# Autodesk Inventor assembly: 6001JRXZZ
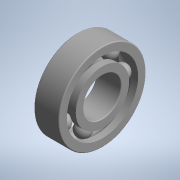
[picture p0: Inventor's stored thumbnail of the model, 180x180]
Saved by Autodesk Inventor 2022.3 (Build 263350000, 350)
## iProperties
Part Number: 6001JRXZZ
Catalog Web Link: www.cadenas.de
Description: Shielded type ZZ-
Vendor: NTN
Document SubType Name: Assembly
Designer: partserver
Manufacturer: NTN
Mass: 2.63039 g
Surface Area: 31.8837 cm^2
Volume: 2.63039 cm^3
Density: 1 g/cm^3
Category: PARTsolutions
Company: NTN
PSOL_IDENT_0: {$CADENAS_DATA\23d-libs\ntn\ball_roller_bearings\deep_groove_bb\deep_groove_bb\dgbb_zz_asmtab.prj},1
PSOL_IDENT_1: 84 {VTYP=3D},{STYP=ASSTAB},{NB=6001JRXZZ},{LINA=6001JRXZZ},{NN=Shielded type ZZ},{DATE=12.08.2020 02
PSOL_IDENT_2: :23:38},{GEOMDATE=29.05.2020 01:04:27},{VERSION=},{LINEID=8380},{WBVAR=},{WBNUMERIC=}  {NB=6001JRXZZ
PSOL_IDENT_3: },{LINA=6001JRXZZ},{KT=DUMMY},{IDNR=},{SD=12},{D=28},{B=8},{R=0.3},{ORDER1=6001JRX},{ORDER=6001JRXZZ
PSOL_IDENT_4: },{CR=5.65},{COR=2.39},{CU=0.3},{CRF=MIN},{CORF=MIN},{LSG=26000},{LSO=30000},{MASS=0.021},{RNS=MIN},
PSOL_IDENT_5: {LLH=MIN},{LLU=MIN},{ST=},{NCST=},{LTST=},{CST=},{SRG=},{SR=},{D1=26.44},{A=2.20},{BA=0.90},{R0=0.30
PSOL_IDENT_6: },{D2=32.7},{F=MIN},{DA1=},{DA2=},{DA=},{DX=MIN},{CY=},{CZ=},{RAS=},{RNAS=0.182},{VERS=2},{X=8},{PPA
PSOL_IDENT_7: TH=dgbb_asmtpl.prj},{RDX=2},{RD=1}
NB: 6001JRXZZ
NN: Shielded type ZZ
NBSYN: $ORDER.
LINA: 6001JRXZZ
CATALOG: NTN Corporation
SD: 12
D: 28
B: 8
R: 0.3
ORDER: 6001JRXZZ
CR: 5.65
COR: 2.39
CU: 0.3
LSG: 26000
LSO: 30000
MASS: 0.021
SUPPLIER: NTN
ARTICLENO: 6001JRXZZ
BOMINFO: 6001JRXZZ
CREATOR: CADENAS GmbH
Title: 6001JRXZZ
Author: Cadenas PARTsolutions
## Documents named in this file (4)
- C:\Users\YusukeKunita\Documents\GrabCAD\Development\BasicParts\Bearing\NTN_6001JRXZZ\6001JRXZZ.iam
- C:\Users\YusukeKunita\Documents\GrabCAD\Development\BasicParts\Bearing\NTN_6001JRXZZ\6001JRX Inner Ring.ipt
- C:\Users\YusukeKunita\Documents\GrabCAD\Development\BasicParts\Bearing\NTN_6001JRXZZ\6001JRX Outer Ring.ipt
- C:\Users\YusukeKunita\Documents\GrabCAD\Development\BasicParts\Bearing\NTN_6001JRXZZ\6001JRX Ball.ipt
## Components (9 placed, 3 different names)
1. 6001JRX Inner Ring:1 — dgbb_ir_XY@1 <-> dgbb_or_XY@2, dgbb_ir_Z@1 <-> dgbb_or_Z@2, dgbb_ir_YZ@1 <-> dgbb_or_YZ@2
2. 6001JRX Outer Ring:1 — dgbb_ir_XY@1 <-> dgbb_or_XY@2, dgbb_ir_Z@1 <-> dgbb_or_Z@2, dgbb_ir_YZ@1 <-> dgbb_or_YZ@2, dgbb_or11_1_XY@2 <-> dgbb_ball_XY@3, dgbb_or11_1_Z@2 <-> dgbb_ball_Z@3, dgbb_or11_1_YZ@2 <-> dgbb_ball_YZ@3, dgbb_or11_2_XY@2 <-> dgbb_ball_XY@4, dgbb_or11_2_Z@2 <-> dgbb_ball_Z@4, dgbb_or11_2_YZ@2 <-> dgbb_ball_YZ@4, dgbb_or11_3_XY@2 <-> dgbb_ball_XY@5, dgbb_or11_3_Z@2 <-> dgbb_ball_Z@5, dgbb_or11_3_YZ@2 <-> dgbb_ball_YZ@5, dgbb_or11_4_XY@2 <-> dgbb_ball_XY@6, dgbb_or11_4_Z@2 <-> dgbb_ball_Z@6, dgbb_or11_4_YZ@2 <-> dgbb_ball_YZ@6, dgbb_or11_5_XY@2 <-> dgbb_ball_XY@7, dgbb_or11_5_Z@2 <-> dgbb_ball_Z@7, dgbb_or11_5_YZ@2 <-> dgbb_ball_YZ@7, dgbb_or11_6_XY@2 <-> dgbb_ball_XY@8, dgbb_or11_6_Z@2 <-> dgbb_ball_Z@8, dgbb_or11_6_YZ@2 <-> dgbb_ball_YZ@8, dgbb_or11_7_XY@2 <-> dgbb_ball_XY@9, dgbb_or11_7_Z@2 <-> dgbb_ball_Z@9, dgbb_or11_7_YZ@2 <-> dgbb_ball_YZ@9
3. 6001JRX Ball:1 — dgbb_or11_1_XY@2 <-> dgbb_ball_XY@3, dgbb_or11_1_Z@2 <-> dgbb_ball_Z@3, dgbb_or11_1_YZ@2 <-> dgbb_ball_YZ@3
4. 6001JRX Ball:2 — dgbb_or11_2_XY@2 <-> dgbb_ball_XY@4, dgbb_or11_2_Z@2 <-> dgbb_ball_Z@4, dgbb_or11_2_YZ@2 <-> dgbb_ball_YZ@4
5. 6001JRX Ball:3 — dgbb_or11_3_XY@2 <-> dgbb_ball_XY@5, dgbb_or11_3_Z@2 <-> dgbb_ball_Z@5, dgbb_or11_3_YZ@2 <-> dgbb_ball_YZ@5
6. 6001JRX Ball:4 — dgbb_or11_4_XY@2 <-> dgbb_ball_XY@6, dgbb_or11_4_Z@2 <-> dgbb_ball_Z@6, dgbb_or11_4_YZ@2 <-> dgbb_ball_YZ@6
7. 6001JRX Ball:5 — dgbb_or11_5_XY@2 <-> dgbb_ball_XY@7, dgbb_or11_5_Z@2 <-> dgbb_ball_Z@7, dgbb_or11_5_YZ@2 <-> dgbb_ball_YZ@7
8. 6001JRX Ball:6 — dgbb_or11_6_XY@2 <-> dgbb_ball_XY@8, dgbb_or11_6_Z@2 <-> dgbb_ball_Z@8, dgbb_or11_6_YZ@2 <-> dgbb_ball_YZ@8
9. 6001JRX Ball:7 — dgbb_or11_7_XY@2 <-> dgbb_ball_XY@9, dgbb_or11_7_Z@2 <-> dgbb_ball_Z@9, dgbb_or11_7_YZ@2 <-> dgbb_ball_YZ@9
## Relationships (24: Mate 15, Angle 8, Flush 1)
- dgbb_ir_XY@1 <-> dgbb_or_XY@2 [Flush]: 6001JRX Inner Ring:1 ↔ 6001JRX Outer Ring:1
- dgbb_ir_Z@1 <-> dgbb_or_Z@2 [Mate]: 6001JRX Inner Ring:1 ↔ 6001JRX Outer Ring:1
- dgbb_ir_YZ@1 <-> dgbb_or_YZ@2 [Angle] (0 deg): 6001JRX Inner Ring:1 ↔ 6001JRX Outer Ring:1
- dgbb_or11_1_XY@2 <-> dgbb_ball_XY@3 [Mate]: 6001JRX Outer Ring:1 ↔ 6001JRX Ball:1
- dgbb_or11_1_Z@2 <-> dgbb_ball_Z@3 [Mate]: 6001JRX Outer Ring:1 ↔ 6001JRX Ball:1
- dgbb_or11_1_YZ@2 <-> dgbb_ball_YZ@3 [Angle] (0 deg): 6001JRX Outer Ring:1 ↔ 6001JRX Ball:1
- dgbb_or11_2_XY@2 <-> dgbb_ball_XY@4 [Mate]: 6001JRX Outer Ring:1 ↔ 6001JRX Ball:2
- dgbb_or11_2_Z@2 <-> dgbb_ball_Z@4 [Mate]: 6001JRX Outer Ring:1 ↔ 6001JRX Ball:2
- dgbb_or11_2_YZ@2 <-> dgbb_ball_YZ@4 [Angle] (0 deg): 6001JRX Outer Ring:1 ↔ 6001JRX Ball:2
- dgbb_or11_3_XY@2 <-> dgbb_ball_XY@5 [Mate]: 6001JRX Outer Ring:1 ↔ 6001JRX Ball:3
- dgbb_or11_3_Z@2 <-> dgbb_ball_Z@5 [Mate]: 6001JRX Outer Ring:1 ↔ 6001JRX Ball:3
- dgbb_or11_3_YZ@2 <-> dgbb_ball_YZ@5 [Angle] (0 deg): 6001JRX Outer Ring:1 ↔ 6001JRX Ball:3
- dgbb_or11_4_XY@2 <-> dgbb_ball_XY@6 [Mate]: 6001JRX Outer Ring:1 ↔ 6001JRX Ball:4
- dgbb_or11_4_Z@2 <-> dgbb_ball_Z@6 [Mate]: 6001JRX Outer Ring:1 ↔ 6001JRX Ball:4
- dgbb_or11_4_YZ@2 <-> dgbb_ball_YZ@6 [Angle] (0 deg): 6001JRX Outer Ring:1 ↔ 6001JRX Ball:4
- dgbb_or11_5_XY@2 <-> dgbb_ball_XY@7 [Mate]: 6001JRX Outer Ring:1 ↔ 6001JRX Ball:5
- dgbb_or11_5_Z@2 <-> dgbb_ball_Z@7 [Mate]: 6001JRX Outer Ring:1 ↔ 6001JRX Ball:5
- dgbb_or11_5_YZ@2 <-> dgbb_ball_YZ@7 [Angle] (0 deg): 6001JRX Outer Ring:1 ↔ 6001JRX Ball:5
- dgbb_or11_6_XY@2 <-> dgbb_ball_XY@8 [Mate]: 6001JRX Outer Ring:1 ↔ 6001JRX Ball:6
- dgbb_or11_6_Z@2 <-> dgbb_ball_Z@8 [Mate]: 6001JRX Outer Ring:1 ↔ 6001JRX Ball:6
- dgbb_or11_6_YZ@2 <-> dgbb_ball_YZ@8 [Angle] (0 deg): 6001JRX Outer Ring:1 ↔ 6001JRX Ball:6
- dgbb_or11_7_XY@2 <-> dgbb_ball_XY@9 [Mate]: 6001JRX Outer Ring:1 ↔ 6001JRX Ball:7
- dgbb_or11_7_Z@2 <-> dgbb_ball_Z@9 [Mate]: 6001JRX Outer Ring:1 ↔ 6001JRX Ball:7
- dgbb_or11_7_YZ@2 <-> dgbb_ball_YZ@9 [Angle] (0 deg): 6001JRX Outer Ring:1 ↔ 6001JRX Ball:7
